# Autodesk Inventor assembly: MultiPass100V-0V-Overlap-V2
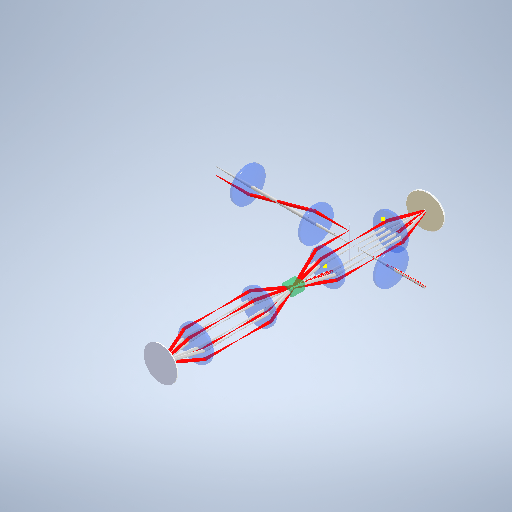
[picture p0: Inventor's stored thumbnail of the model, 512x512]
Saved by Autodesk Inventor 2025 (Build 290162010, 162A)
## iProperties
Created: 2024-09-03
Part Number: MultiPass100V-0V-Overlap-V2
Document SubType Name: Assembly
Designer: User
Author: User
## Documents named in this file (3)
- C:\Users\User\Desktop\Hari_Laptop_Contents\KerlinLab\KTN\Multipass\MechanicalDrawing\MultiPass100V-0V-Overlap-V2.iam
- C:\Users\User\Desktop\Hari_Laptop_Contents\KerlinLab\KTN\Multipass\MechanicalDrawing\MultiPass100V.iam
- C:\Users\User\Desktop\Hari_Laptop_Contents\KerlinLab\KTN\Multipass\MechanicalDrawing\MultiPass0V-OnlyRays-V2.iam
## Components (2 placed, 2 different names)
1. MultiPass100V:1 [sub-assembly] — Mate:1, Mate:2
2. MultiPass0V-OnlyRays-V2:1 [sub-assembly] — Mate:1, Mate:2
## Relationships (2: Mate 2)
- Mate:1: MultiPass100V:1 ↔ MultiPass0V-OnlyRays-V2:1
- Mate:2: MultiPass100V:1 ↔ MultiPass0V-OnlyRays-V2:1
